# Autodesk Inventor assembly: assem
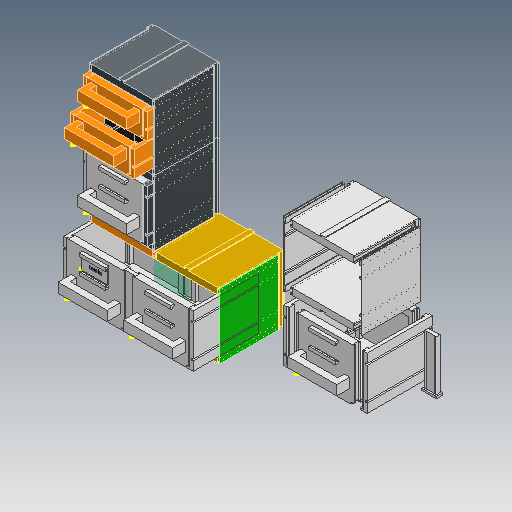
[picture p0: Inventor's stored thumbnail of the model, 512x512]
Saved by Autodesk Inventor 2025.2 (Build 292293000, 293)
## iProperties
Created: 2025-02-22
Part Number: assem
Document SubType Name: Assembly
Designer: email
Author: email
## Documents named in this file (9)
- C:\Users\email\Desktop\Projects\modularboxes\V1\assem.iam
- C:\Users\email\Desktop\Projects\modularboxes\V1\mainframe.ipt
- C:\Users\email\Desktop\Projects\modularboxes\V1\side.ipt
- C:\Users\email\Desktop\Projects\modularboxes\V1\drawerside.ipt
- C:\Users\email\Desktop\Projects\modularboxes\V1\maindrawer.ipt
- C:\Users\email\Desktop\Projects\modularboxes\V1\drawerconnector.ipt
- C:\Users\email\Desktop\Projects\modularboxes\V1\boxassem.iam
- C:\Users\email\Desktop\Projects\modularboxes\V1\halfdrawerassem.iam
- C:\Users\email\Desktop\Projects\modularboxes\V1\drawersign.ipt
## Components (29 placed, 8 different names)
1. mainframe:2 — Mate:1, Mate:2, Mate:3, Mate:4, Mate:5, Mate:6, Mate:7, Mate:14, Flush:1, Mate:15, Mate:16, Flush:2
2. mainframe:3 — Mate:7, Mate:8, Mate:9, Mate:10, Mate:11, Mate:12, Mate:13, Mate:14, Flush:1, Mate:65
3. mainframe:4 — Mate:15, Mate:16, Flush:2, Mate:17, Mate:18, Mate:19, Mate:20, Mate:21, Mate:22, Mate:31, Mate:55, Mate:56, Flush:3
4. side:1 — Mate:1, Mate:2, Mate:5, Mate:47, Mate:48
5. side:2 — Mate:3, Mate:4, Mate:6
6. side:3 — Mate:8, Mate:9, Mate:12
7. side:4 — Mate:10, Mate:11, Mate:13
8. side:5 — Mate:17, Mate:18, Mate:22, Mate:29, Mate:30
9. side:6 — Mate:19, Mate:20, Mate:21
10. drawerside:1 — Mate:23, Mate:24, Mate:25, Mate:29, Mate:30
11. maindrawer:1 — Mate:23, Mate:24, Mate:25, Mate:26, Mate:27, Mate:28, Mate:31
12. drawerside:2 — Mate:26, Mate:27, Mate:28
13. maindrawer:2 — Mate:32, Mate:33, Mate:34, Mate:38, Mate:39, Mate:40, Mate:44, Mate:46, Mate:63, Mate:64, Flush:4
14. drawerside:3 — Mate:35, Mate:36, Mate:37
15. drawerside:4 — Mate:32, Mate:33, Mate:34, Mate:47, Mate:48
16. maindrawer:3 — Mate:35, Mate:36, Mate:37, Mate:41, Mate:42, Mate:43, Mate:45, Mate:65
17. drawerconnector:2 — Mate:38, Mate:39, Mate:40, Mate:41, Mate:42, Mate:43
18. drawerconnector:3 — Mate:44, Mate:45, Mate:46
19. drawerconnector:4
20. maindrawer:4 — Flush:70, Flush:71, Mate:69, Mate:70, Flush:72, Mate:71
21. drawerside:5 — Flush:70, Flush:71, Mate:69
22. drawerside:6 — Mate:70, Flush:72, Mate:71
23. mainframe:5 — Mate:66, Flush:5, Flush:6, Mate:67, Flush:7, Mate:68
24. side:7 — Mate:66, Flush:5, Flush:6
25. side:8 — Mate:67, Flush:7, Mate:68
26. boxassem:1 [sub-assembly] — Mate:55, Mate:56, Flush:3, Mate:57, Mate:58, Mate:59, Mate:60, Mate:61, Mate:62
27. halfdrawerassem:1 [sub-assembly] — Mate:57, Mate:58, Mate:59
28. halfdrawerassem:2 [sub-assembly] — Mate:60, Mate:61, Mate:62
29. drawersign:1 — Mate:63, Mate:64, Flush:4
## Relationships (75: Mate 65, Flush 10)
- Mate:1: mainframe:2 ↔ side:1
- Mate:2: mainframe:2 ↔ side:1
- Mate:3: mainframe:2 ↔ side:2
- Mate:4: mainframe:2 ↔ side:2
- Mate:5: mainframe:2 ↔ side:1
- Mate:6: mainframe:2 ↔ side:2
- Mate:7: mainframe:2 ↔ mainframe:3
- Mate:8: mainframe:3 ↔ side:3
- Mate:9: mainframe:3 ↔ side:3
- Mate:10: mainframe:3 ↔ side:4
- Mate:11: mainframe:3 ↔ side:4
- Mate:12: mainframe:3 ↔ side:3
- Mate:13: mainframe:3 ↔ side:4
- Mate:14: mainframe:2 ↔ mainframe:3
- Flush:1: mainframe:2 ↔ mainframe:3
- Mate:15: mainframe:2 ↔ mainframe:4
- Mate:16: mainframe:2 ↔ mainframe:4
- Flush:2: mainframe:2 ↔ mainframe:4
- Mate:17: mainframe:4 ↔ side:5
- Mate:18: mainframe:4 ↔ side:5
- Mate:19: mainframe:4 ↔ side:6
- Mate:20: mainframe:4 ↔ side:6
- Mate:21: mainframe:4 ↔ side:6
- Mate:22: mainframe:4 ↔ side:5
- Mate:23: drawerside:1 ↔ maindrawer:1
- Mate:24: drawerside:1 ↔ maindrawer:1
- Mate:25: drawerside:1 ↔ maindrawer:1
- Mate:26: maindrawer:1 ↔ drawerside:2
- Mate:27: maindrawer:1 ↔ drawerside:2
- Mate:28: maindrawer:1 ↔ drawerside:2
- Mate:29: side:5 ↔ drawerside:1
- Mate:30: side:5 ↔ drawerside:1
- Mate:31: mainframe:4 ↔ maindrawer:1
- Mate:32: maindrawer:2 ↔ drawerside:4
- Mate:33: maindrawer:2 ↔ drawerside:4
- Mate:34: maindrawer:2 ↔ drawerside:4
- Mate:35: drawerside:3 ↔ maindrawer:3
- Mate:36: drawerside:3 ↔ maindrawer:3
- Mate:37: drawerside:3 ↔ maindrawer:3
- Mate:38: maindrawer:2 ↔ drawerconnector:2
- Mate:39: maindrawer:2 ↔ drawerconnector:2
- Mate:40: maindrawer:2 ↔ drawerconnector:2
- Mate:41: maindrawer:3 ↔ drawerconnector:2
- Mate:42: maindrawer:3 ↔ drawerconnector:2
- Mate:43: maindrawer:3 ↔ drawerconnector:2
- Mate:44: maindrawer:2 ↔ drawerconnector:3
- Mate:45: maindrawer:3 ↔ drawerconnector:3
- Mate:46: maindrawer:2 ↔ drawerconnector:3
- Mate:47: side:1 ↔ drawerside:4
- Mate:48: side:1 ↔ drawerside:4
- Mate:55: mainframe:4 ↔ boxassem:1
- Mate:56: mainframe:4 ↔ boxassem:1
- Flush:3: mainframe:4 ↔ boxassem:1
- Mate:57: boxassem:1 ↔ halfdrawerassem:1
- Mate:58: boxassem:1 ↔ halfdrawerassem:1
- Mate:59 (20 mm): boxassem:1 ↔ halfdrawerassem:1
- Mate:60: boxassem:1 ↔ halfdrawerassem:2
- Mate:61 (-10 mm): boxassem:1 ↔ halfdrawerassem:2
- Mate:62: boxassem:1 ↔ halfdrawerassem:2
- Mate:63: maindrawer:2 ↔ drawersign:1
- Mate:64: maindrawer:2 ↔ drawersign:1
- Flush:4: maindrawer:2 ↔ drawersign:1
- Mate:65 (30 mm): mainframe:3 ↔ maindrawer:3
- Mate:66 (10 mm): mainframe:5 ↔ side:7
- Flush:5: mainframe:5 ↔ side:7
- Flush:6: mainframe:5 ↔ side:7
- Mate:67 (10 mm): mainframe:5 ↔ side:8
- Flush:7: mainframe:5 ↔ side:8
- Mate:68: mainframe:5 ↔ side:8
- Flush:70: maindrawer:4 ↔ drawerside:5
- Flush:71: maindrawer:4 ↔ drawerside:5
- Mate:69 (15 mm): maindrawer:4 ↔ drawerside:5
- Mate:70 (15 mm): maindrawer:4 ↔ drawerside:6
- Flush:72: maindrawer:4 ↔ drawerside:6
- Mate:71: maindrawer:4 ↔ drawerside:6
